# Autodesk Inventor assembly: slider assembly
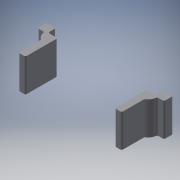
[picture p0: Inventor's stored thumbnail of the model, 180x180]
Saved by Autodesk Inventor 2016 (Build 200138000, 138)
## iProperties
Created: 2016-02-14
Part Number: slider assembly
Document SubType Name: Assembly
Designer: Margret
Author: Margret
## Documents named in this file (2)
- C:\Users\Margret\Documents\Inventor\igus slider cap\slider assembly.iam
- C:\Users\Margret\Documents\Inventor\igus slider cap\Igus Slider.ipt
## Components (2 placed, 1 different names)
1. Igus Slider:1 — Flush:1, Flush:2, Mate:1
2. Igus Slider:2 — Flush:1, Flush:2, Mate:1
## Relationships (3: Flush 2, Mate 1)
- Flush:1: Igus Slider:1 ↔ Igus Slider:2
- Flush:2: Igus Slider:1 ↔ Igus Slider:2
- Mate:1 (68.7324 mm): Igus Slider:1 ↔ Igus Slider:2
